# Autodesk Inventor assembly: Ensamblaje José Palacios
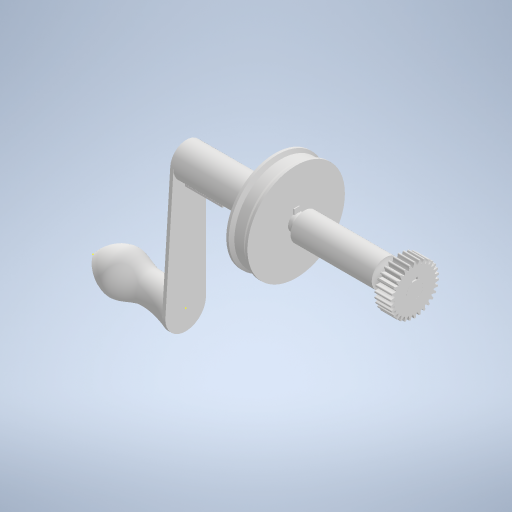
[picture p0: Inventor's stored thumbnail of the model, 512x512]
Saved by Autodesk Inventor 2024.2 (Build 282272000, 272)
## iProperties
Created: 2024-03-18
Part Number: Ensamblaje José Palacios
Document SubType Name: Assembly
Designer: josep
Author: josep
## Documents named in this file (6)
- C:\Users\josep\OneDrive\Documents\URL Ingeniería\Ciclo 2024\I Semestre\Dinámica\Lab Dinamica\Inventor\Ensamblaje José Palacios.iam
- C:\Users\josep\Downloads\CUÑA (1).ipt
- C:\Users\josep\Downloads\EJE_CUÑEROS.ipt
- C:\Users\josep\Downloads\POLEA.ipt
- C:\Users\josep\Downloads\ENGRANE.ipt
- C:\Users\josep\OneDrive\Documents\URL Ingeniería\Ciclo 2024\I Semestre\Dinámica\Lab Dinamica\Inventor\Manivela José Palacios.ipt
## Components (6 placed, 5 different names)
1. EJE_CUÑEROS:1 — Rigid:2, Flush:3, Rigid:3, Rigid:4, Flush:6, Mate:1, Mate:2, Rigid:5, Flush:7, Flush:8, Rotational:1
2. CUÑA (1):1 — Rigid:3, Mate:2
3. CUÑA (1):2 — Rigid:2, Flush:3, Mate:1
4. POLEA:1 — Rigid:4, Flush:6, Flush:9
5. ENGRANE:1 — Rigid:5, Flush:7, Flush:8
6. Manivela José Palacios:1 — Rotational:1, Flush:9
## Relationships (12: Flush 5, WeldJoint 4, Mate 2, RevoluteJoint 1)
- Rigid:2 [WeldJoint]: EJE_CUÑEROS:1 ↔ CUÑA (1):2
- Flush:3: EJE_CUÑEROS:1 ↔ CUÑA (1):2
- Rigid:3 [WeldJoint]: EJE_CUÑEROS:1 ↔ CUÑA (1):1
- Rigid:4 [WeldJoint]: EJE_CUÑEROS:1 ↔ POLEA:1
- Flush:6: EJE_CUÑEROS:1 ↔ POLEA:1
- Mate:1: EJE_CUÑEROS:1 ↔ CUÑA (1):2
- Mate:2: EJE_CUÑEROS:1 ↔ CUÑA (1):1
- Rigid:5 [WeldJoint]: EJE_CUÑEROS:1 ↔ ENGRANE:1
- Flush:7: EJE_CUÑEROS:1 ↔ ENGRANE:1
- Flush:8: EJE_CUÑEROS:1 ↔ ENGRANE:1
- Rotational:1 [RevoluteJoint]: EJE_CUÑEROS:1 ↔ Manivela José Palacios:1
- Flush:9: POLEA:1 ↔ Manivela José Palacios:1
